# Autodesk Inventor assembly: Apogee Sherpa Full
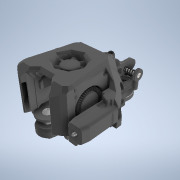
[picture p0: Inventor's stored thumbnail of the model, 180x180]
Saved by Autodesk Inventor 2022 (Build 260153000, 153)
## iProperties
Created: 2023-12-26
Part Number: Apogee Sherpa Full
Document SubType Name: Assembly
Designer: Admin
Author: Admin
## Documents named in this file (11)
- C:\Users\Admin\Documents\GitHub\ApogeeSherpa\Apogee Sherpa Full.iam
- C:\Users\Admin\Documents\GitHub\ApogeeSherpa\X_Carriage\Ender 3 V2 X Carriage.iam
- C:\Users\Admin\Documents\GitHub\ApogeeSherpa\ApogeeSherpa\SH_HotendBase_Volcano.ipt
- C:\Users\Admin\Documents\GitHub\ApogeeSherpa\Volcano\Volcano Hotend.iam
- C:\Users\Admin\Documents\GitHub\ApogeeSherpa\ApogeeSherpa\SH_CR_Touch-Holder v3.ipt
- C:\Users\Admin\Documents\GitHub\ApogeeSherpa\ApogeeSherpa\CR-Touch-Dummy v1.ipt
- C:\Users\Admin\Documents\GitHub\ApogeeSherpa\SherpaMini\sherpa_mini_release_2.iam
- C:\Users\Admin\Documents\GitHub\ApogeeSherpa\ApogeeSherpa\SH_Wire-Cover v1.ipt
- C:\Users\Admin\Documents\GitHub\ApogeeSherpa\ApogeeSherpa\SH_FanSchroud.ipt
- C:\Users\Admin\Documents\GitHub\ApogeeSherpa\Fans\3010 Fan.ipt
- C:\Users\Admin\Documents\GitHub\ApogeeSherpa\Fans\4010 Fan.ipt
## Components (11 placed, 10 different names)
1. Ender 3 V2 X Carriage:1 [sub-assembly] — Жесткий:1
2. SH_HotendBase_Volcano:1 — Жесткий:1, Жесткий:2, Жесткий:3, Жесткий:5, Жесткий:6, Жесткий:10
3. Volcano Hotend:1 [sub-assembly] — Жесткий:2
4. SH_CR_Touch-Holder v3:1 — Жесткий:3, Жесткий:4
5. CR-Touch-Dummy v1:1 — Жесткий:4
6. sherpa_mini_release_2:1 [sub-assembly] — Жесткий:5
7. SH_Wire-Cover v1:1 — Жесткий:6
8. SH_FanSchroud:1 — Жесткий:7, Жесткий:8, Жесткий:9, Жесткий:10
9. 3010 Fan:1 — Жесткий:7
10. 4010 Fan:1 — Жесткий:9
11. 4010 Fan:2 — Жесткий:8
## Relationships (10: WeldJoint 10)
- Жесткий:1 [WeldJoint]: Ender 3 V2 X Carriage:1 ↔ SH_HotendBase_Volcano:1
- Жесткий:2 [WeldJoint]: SH_HotendBase_Volcano:1 ↔ Volcano Hotend:1
- Жесткий:3 [WeldJoint]: SH_HotendBase_Volcano:1 ↔ SH_CR_Touch-Holder v3:1
- Жесткий:4 [WeldJoint]: SH_CR_Touch-Holder v3:1 ↔ CR-Touch-Dummy v1:1
- Жесткий:5 [WeldJoint]: SH_HotendBase_Volcano:1 ↔ sherpa_mini_release_2:1
- Жесткий:6 [WeldJoint]: SH_HotendBase_Volcano:1 ↔ SH_Wire-Cover v1:1
- Жесткий:7 [WeldJoint]: SH_FanSchroud:1 ↔ 3010 Fan:1
- Жесткий:8 [WeldJoint]: SH_FanSchroud:1 ↔ 4010 Fan:2
- Жесткий:9 [WeldJoint]: SH_FanSchroud:1 ↔ 4010 Fan:1
- Жесткий:10 [WeldJoint]: SH_HotendBase_Volcano:1 ↔ SH_FanSchroud:1
